# Autodesk Inventor assembly: R-Upright2018
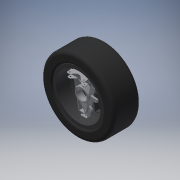
[picture p0: Inventor's stored thumbnail of the model, 180x180]
Saved by Autodesk Inventor 2018.2 (Build 222227000, 227)
## iProperties
Created: 2018-05-19
Part Number: R-Upright2018
Material: 一般
Document SubType Name: Assembly
Designer: ku_sk
Sending System: Autodesk Inventor 2018
Preprocessor: ST-DEVELOPER v17
Title: D:\ku_sk\ドキュメント\Inventor\Aero\KS-15\全体アッセンブリ解析用モデル\body\sus\R-Upright2018.stp
Author: ku_sk
## Documents named in this file (5)
- D:\ku_sk\ドキュメント\Inventor\Aero\KS-15\全体アッセンブリ解析用モデル\body\sus\R-Upright2018.iam
- D:\ku_sk\ドキュメント\Inventor\Aero\KS-15\全体アッセンブリ解析用モデル\body\sus\Rear Upright 4.16.ipt
- D:\ku_sk\ドキュメント\Inventor\Aero\KS-15\全体アッセンブリ解析用モデル\body\sus\R-Upright Bracket 2018.ipt
- D:\ku_sk\ドキュメント\Inventor\Aero\KS-15\全体アッセンブリ解析用モデル\body\sus\R-Sim13 2018.ipt
- D:\ku_sk\ドキュメント\Inventor\Aero\KS-15\全体アッセンブリ解析用モデル\body\sus\2015Wheel watanabe.ipt
## Components (4 placed, 4 different names)
1. Rear Upright 4.16.1 — メイト:1, メイト:2
2. R-Upright Bracket 2018.1
3. R-Sim13 2018.1
4. 2015Wheel watanabe:1 — メイト:1, メイト:2
## Relationships (2: Mate 2)
- メイト:1 [Mate]: Rear Upright 4.16.1 ↔ 2015Wheel watanabe:1
- メイト:2 [Mate] (49 mm): Rear Upright 4.16.1 ↔ 2015Wheel watanabe:1
